# Autodesk Inventor assembly: Cart_Chassis
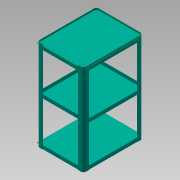
[picture p0: Inventor's stored thumbnail of the model, 180x180]
Saved by Autodesk Inventor 2015 (Build 190159000, 159)
## iProperties
Created: 2015-05-21
Part Number: Cart_Chassis
Document SubType Name: Assembly
Designer: Joe Sheldon
Author: Joe Sheldon
## Documents named in this file (6)
- C:\Users\Joe Sheldon\Documents\PSU Stuff\PSU Clubs\Society of Physics Students\Cloud Chamber\Cloud Chamber CAD\Cart_Chassis.iam
- C:\Users\Joe Sheldon\Documents\PSU Stuff\PSU Clubs\Society of Physics Students\Cloud Chamber\Cloud Chamber CAD\Cart_LOW_SHELF.ipt
- C:\Users\Joe Sheldon\Documents\PSU Stuff\PSU Clubs\Society of Physics Students\Cloud Chamber\Cloud Chamber CAD\Cart_MID_SHELF.ipt
- C:\Users\Joe Sheldon\Documents\PSU Stuff\PSU Clubs\Society of Physics Students\Cloud Chamber\Cloud Chamber CAD\Cart_TOP_SHELF.ipt
- C:\Users\Joe Sheldon\Documents\PSU Stuff\PSU Clubs\Society of Physics Students\Cloud Chamber\Cloud Chamber CAD\Cart_Side_Beam.ipt
- C:\Users\Joe Sheldon\Documents\PSU Stuff\PSU Clubs\Society of Physics Students\Cloud Chamber\Cloud Chamber CAD\Cart_TOP_SHELF-LIP.ipt
## Components (8 placed, 5 different names)
1. Cart_LOW_SHELF:1 — Rigid:1, Rigid:2, Rigid:3, Rigid:4
2. Cart_MID_SHELF:1 — Rigid:6
3. Cart_TOP_SHELF:1 — Rigid:5
4. Cart_Side_Beam:1 — Rigid:3
5. Cart_Side_Beam:2 — Rigid:1
6. Cart_Side_Beam:3 — Rigid:2, Rigid:5, Rigid:6, Rigid:7
7. Cart_Side_Beam:4 — Rigid:4
8. Cart_TOP_SHELF-LIP:1 — Rigid:7
## Relationships (7: WeldJoint 7)
- Rigid:1 [WeldJoint]: Cart_LOW_SHELF:1 ↔ Cart_Side_Beam:2
- Rigid:2 [WeldJoint]: Cart_LOW_SHELF:1 ↔ Cart_Side_Beam:3
- Rigid:3 [WeldJoint]: Cart_LOW_SHELF:1 ↔ Cart_Side_Beam:1
- Rigid:4 [WeldJoint]: Cart_LOW_SHELF:1 ↔ Cart_Side_Beam:4
- Rigid:5 [WeldJoint] (2.8448 mm): Cart_TOP_SHELF:1 ↔ Cart_Side_Beam:3
- Rigid:6 [WeldJoint] (355.6 mm): Cart_MID_SHELF:1 ↔ Cart_Side_Beam:3
- Rigid:7 [WeldJoint] (12.7 mm): Cart_Side_Beam:3 ↔ Cart_TOP_SHELF-LIP:1
